# Autodesk Inventor assembly: rover-encoder-assembly
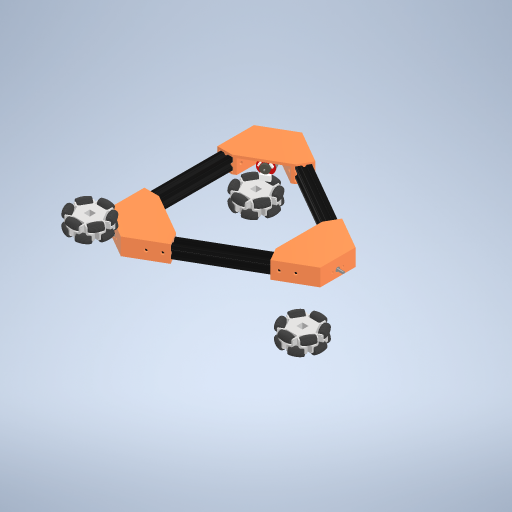
[picture p0: Inventor's stored thumbnail of the model, 512x512]
Saved by Autodesk Inventor 2024.2 (Build 282272000, 272)
## iProperties
Created: 2024-04-23
Part Number: rover-encoder-assembly
Document SubType Name: Assembly
Designer: Robin
Author: Robin
## Documents named in this file (5)
- C:\Users\Robin\OneDrive\Study\Current\Mechanical Design\Cad\fork-cad\rover-encoder-assembly.iam
- C:\Users\Robin\OneDrive\Study\Current\Mechanical Design\Cad\fork-cad\cornerBracket_Encoder.ipt
- C:\Users\Robin\OneDrive\Study\Current\Mechanical Design\Cad\fork-cad\2020aluminum_extrusion_black.ipt
- C:\Users\Robin\OneDrive\Study\Current\Mechanical Design\Cad\fork-cad\JGA25-370 DC12V350RPM\JGA25-370 DC12V350RPM.ipt
- C:\Users\Robin\OneDrive\Study\Current\Mechanical Design\Cad\fork-cad\wheel-assembly.iam
## Components (12 placed, 4 different names)
1. cornerBracket_Encoder:1 — Mate:1, Mate:2, Mate:3, Mate:4, Mate:5, Mate:6, Mate:18, Mate:19
2. cornerBracket_Encoder:2 — Mate:10, Mate:11, Mate:12, Mate:13, Mate:14, Mate:15, Mate:17, Mate:20
3. cornerBracket_Encoder:3 — Mate:7, Mate:8, Mate:9, Mate:16, Mate:21
4. 2020aluminum_extrusion_black:1 — Mate:11, Mate:12, Mate:13
5. 2020aluminum_extrusion_black:2 — Mate:4, Mate:5, Mate:6, Mate:7, Mate:8, Mate:9
6. 2020aluminum_extrusion_black:3 — Mate:1, Mate:2, Mate:3, Mate:10, Mate:14, Mate:15
7. JGA25-370 DC12V350RPM:1 — Mate:17, Mate:20
8. JGA25-370 DC12V350RPM:2 — Mate:16, Mate:21
9. JGA25-370 DC12V350RPM:3 — Mate:18, Mate:19
10. wheel-assembly:1 [sub-assembly]
11. wheel-assembly:2 [sub-assembly]
12. wheel-assembly:3 [sub-assembly]
## Relationships (21: Mate 21)
- Mate:1: cornerBracket_Encoder:1 ↔ 2020aluminum_extrusion_black:3
- Mate:2 (0.5 mm): cornerBracket_Encoder:1 ↔ 2020aluminum_extrusion_black:3
- Mate:3 (0.5 mm): cornerBracket_Encoder:1 ↔ 2020aluminum_extrusion_black:3
- Mate:4: cornerBracket_Encoder:1 ↔ 2020aluminum_extrusion_black:2
- Mate:5 (0.5 mm): cornerBracket_Encoder:1 ↔ 2020aluminum_extrusion_black:2
- Mate:6 (0.5 mm): cornerBracket_Encoder:1 ↔ 2020aluminum_extrusion_black:2
- Mate:7: cornerBracket_Encoder:3 ↔ 2020aluminum_extrusion_black:2
- Mate:8 (0.5 mm): cornerBracket_Encoder:3 ↔ 2020aluminum_extrusion_black:2
- Mate:9 (0.5 mm): cornerBracket_Encoder:3 ↔ 2020aluminum_extrusion_black:2
- Mate:10: cornerBracket_Encoder:2 ↔ 2020aluminum_extrusion_black:3
- Mate:11: cornerBracket_Encoder:2 ↔ 2020aluminum_extrusion_black:1
- Mate:12 (0.5 mm): cornerBracket_Encoder:2 ↔ 2020aluminum_extrusion_black:1
- Mate:13 (0.5 mm): cornerBracket_Encoder:2 ↔ 2020aluminum_extrusion_black:1
- Mate:14 (0.5 mm): cornerBracket_Encoder:2 ↔ 2020aluminum_extrusion_black:3
- Mate:15 (0.5 mm): cornerBracket_Encoder:2 ↔ 2020aluminum_extrusion_black:3
- Mate:16: cornerBracket_Encoder:3 ↔ JGA25-370 DC12V350RPM:2
- Mate:17: cornerBracket_Encoder:2 ↔ JGA25-370 DC12V350RPM:1
- Mate:18: cornerBracket_Encoder:1 ↔ JGA25-370 DC12V350RPM:3
- Mate:19: cornerBracket_Encoder:1 ↔ JGA25-370 DC12V350RPM:3
- Mate:20: cornerBracket_Encoder:2 ↔ JGA25-370 DC12V350RPM:1
- Mate:21: cornerBracket_Encoder:3 ↔ JGA25-370 DC12V350RPM:2
